# Autodesk Inventor assembly: main room, doors, corridor connected
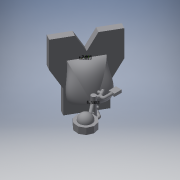
[picture p0: Inventor's stored thumbnail of the model, 180x180]
Saved by Autodesk Inventor 2017 (Build 210142000, 142)
## iProperties
Created: 2018-03-04
Part Number: main room, doors, corridor connected
Document SubType Name: Assembly
Designer: Braxton
Author: Braxton
## Documents named in this file (17)
- D:\School\Game develpment\geoscape\assembly\main room, doors, corridor connected.iam
- D:\School\Game develpment\geoscape\rooms\assembly\main room with double door.iam
- D:\School\Game develpment\geoscape\corridors\corridor.ipt
- D:\School\Game develpment\geoscape\corridors\corridor turn.ipt
- D:\School\Game develpment\geoscape\corridors\T corridor.ipt
- D:\School\Game develpment\geoscape\corridors\Y corridor.ipt
- D:\School\Game develpment\geoscape\corridors\end cap.ipt
- D:\School\Game develpment\geoscape\decoration\table 1 devid 12 size.ipt
- D:\School\Game develpment\geoscape\rooms\dome.ipt
- D:\School\Game develpment\geoscape\corridors\ramp top connect.ipt
- D:\School\Game develpment\geoscape\corridors\ramp.ipt
- D:\School\Game develpment\geoscape\corridors\ramp bottom connect.ipt
- E:\School\Game develpment\geoscape\decoration\terminal.ipt
- D:\School\Game develpment\geoscape\corridors\curve ramp.ipt
- D:\School\Game develpment\geoscape\doors\end door\end door room.ipt
- D:\School\Game develpment\geoscape\doors\end door\assembly\end door assembly.ipt.iam
- end door assembly.ipt
## Components (29 placed, 15 different names)
1. table 1 devid 12 size:1 — Mate:13, Mate:14, Mate:15
2. end door assembly.ipt:1 [sub-assembly] — Flush:26, Flush:27, Mate:21
3. end door room:1 — Flush:26, Flush:27, Mate:21, Flush:34, Insert:33
4. curve ramp:1 — Flush:23, Insert:24, Flush:24, Insert:25, Flush:33, Insert:27, Flush:35, Flush:36, Flush:37, Insert:34, Insert:35, Insert:36, Flush:38, Insert:37
5. ramp top connect:1 — Flush:24, Insert:25, Flush:25, Insert:26
6. corridor turn:2 — Flush:28, Flush:33, Insert:27, Insert:28
7. corridor:3 — Flush:28, Flush:29, Insert:32, Flush:34, Insert:33
8. corridor:4 — Flush:29, Flush:30, Insert:31, Insert:32
9. corridor:5 — Flush:30, Flush:31, Insert:30, Insert:31
10. corridor:6 — Flush:31, Flush:32, Insert:29, Insert:30
11. corridor:7 — Flush:32, Insert:28, Insert:29
12. end cap:2 — Flush:37, Insert:34
13. end cap:3 — Flush:36, Insert:35
14. end cap:4 — Flush:35, Insert:36
15. end cap:5 — Flush:38, Insert:37
16. end cap:6 — Flush:39, Insert:38
17. terminal:1 — Mate:17, Mate:18, Mate:19, Mate:20
18. ramp bottom connect:1 — Flush:19, Insert:18, Flush:22, Insert:23
19. ramp:1 — Flush:17, Insert:20, Flush:25, Insert:26
20. ramp:2 — Flush:17, Flush:18, Insert:19, Insert:20
21. ramp:3 — Flush:18, Flush:19, Insert:18, Insert:19
22. dome:1 — Flush:22, Insert:23, Mate:17, Mate:18, Mate:19, Mate:20
23. main room with double door:1 [sub-assembly] — Mate:13, Mate:14, Mate:15, Flush:1, Insert:1
24. corridor:1 — Flush:1, Flush:2, Insert:1, Insert:2
25. corridor:2 — Flush:2, Flush:3, Insert:2, Insert:3
26. corridor turn:1 — Flush:3, Flush:4, Insert:3, Insert:4
27. Y corridor:1 — Flush:4, Flush:7, Insert:4, Insert:6, Flush:23, Insert:24
28. T corridor:1 — Flush:7, Flush:8, Insert:6, Insert:7, Flush:39, Insert:38
29. end cap:1 — Flush:8, Insert:7
## Relationships (60: Flush 27, Insert 25, Mate 8)
- Mate:13: table 1 devid 12 size:1 ↔ main room with double door:1
- Mate:14 (35.9833 mm): table 1 devid 12 size:1 ↔ main room with double door:1
- Mate:15 (3.175 mm): table 1 devid 12 size:1 ↔ main room with double door:1
- Flush:1: main room with double door:1 ↔ corridor:1
- Flush:2: corridor:1 ↔ corridor:2
- Flush:3: corridor:2 ↔ corridor turn:1
- Flush:4: corridor turn:1 ↔ Y corridor:1
- Flush:7: Y corridor:1 ↔ T corridor:1
- Flush:8: T corridor:1 ↔ end cap:1
- Insert:1: main room with double door:1 ↔ corridor:1
- Insert:2: corridor:1 ↔ corridor:2
- Insert:3: corridor:2 ↔ corridor turn:1
- Insert:4: corridor turn:1 ↔ Y corridor:1
- Insert:6: Y corridor:1 ↔ T corridor:1
- Insert:7: T corridor:1 ↔ end cap:1
- Flush:17: ramp:1 ↔ ramp:2
- Flush:18: ramp:2 ↔ ramp:3
- Flush:19: ramp bottom connect:1 ↔ ramp:3
- Insert:18: ramp bottom connect:1 ↔ ramp:3
- Insert:19: ramp:2 ↔ ramp:3
- Insert:20: ramp:1 ↔ ramp:2
- Flush:22: ramp bottom connect:1 ↔ dome:1
- Insert:23: ramp bottom connect:1 ↔ dome:1
- Mate:17 (762 mm): terminal:1 ↔ dome:1
- Mate:18 (762 mm): terminal:1 ↔ dome:1
- Mate:19: terminal:1 ↔ dome:1
- Mate:20: terminal:1 ↔ dome:1
- Flush:23: curve ramp:1 ↔ Y corridor:1
- Insert:24: curve ramp:1 ↔ Y corridor:1
- Flush:24: curve ramp:1 ↔ ramp top connect:1
- Insert:25: curve ramp:1 ↔ ramp top connect:1
- Flush:25: ramp top connect:1 ↔ ramp:1
- Insert:26: ramp top connect:1 ↔ ramp:1
- Flush:26: end door assembly.ipt:1 ↔ end door room:1
- Flush:27: end door assembly.ipt:1 ↔ end door room:1
- Mate:21: end door assembly.ipt:1 ↔ end door room:1
- Flush:28: corridor turn:2 ↔ corridor:3
- Flush:29: corridor:3 ↔ corridor:4
- Flush:30: corridor:4 ↔ corridor:5
- Flush:31: corridor:5 ↔ corridor:6
- Flush:32: corridor:6 ↔ corridor:7
- Flush:33: curve ramp:1 ↔ corridor turn:2
- Insert:27: curve ramp:1 ↔ corridor turn:2
- Insert:28: corridor turn:2 ↔ corridor:7
- Insert:29: corridor:6 ↔ corridor:7
- Insert:30: corridor:5 ↔ corridor:6
- Insert:31: corridor:4 ↔ corridor:5
- Insert:32: corridor:3 ↔ corridor:4
- Flush:34: end door room:1 ↔ corridor:3
- Insert:33: end door room:1 ↔ corridor:3
- Flush:35: curve ramp:1 ↔ end cap:4
- Flush:36: curve ramp:1 ↔ end cap:3
- Flush:37: curve ramp:1 ↔ end cap:2
- Insert:34: curve ramp:1 ↔ end cap:2
- Insert:35: curve ramp:1 ↔ end cap:3
- Insert:36: curve ramp:1 ↔ end cap:4
- Flush:38: curve ramp:1 ↔ end cap:5
- Insert:37: curve ramp:1 ↔ end cap:5
- Flush:39: end cap:6 ↔ T corridor:1
- Insert:38: end cap:6 ↔ T corridor:1
